# Autodesk Inventor assembly: Hose Assembly
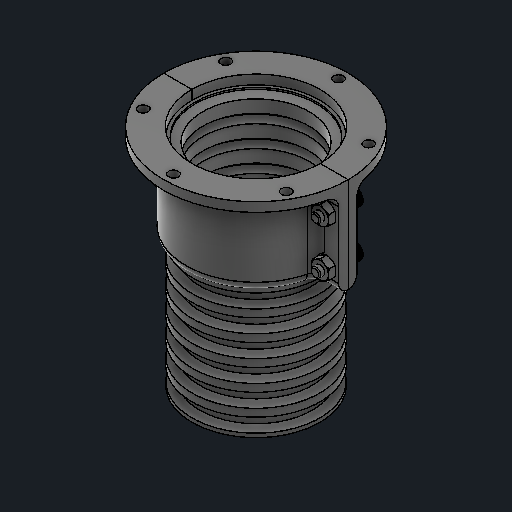
[picture p0: Inventor's stored thumbnail of the model, 512x512]
Saved by Autodesk Inventor 2026.2 (Build 302298000, 298)
## iProperties
Created: 2026-07-12
Part Number: Hose Assembly
Document SubType Name: Assembly
Designer: JoshuaEah
Author: JoshuaEah
## Documents named in this file (5)
- C:\Users\JoshuaEah\Documents\GitHub\Designed-Trinkets\Makera Carvera Air\Air Port\Hose Assembly.iam
- C:\Users\JoshuaEah\Documents\GitHub\Designed-Trinkets\Makera Carvera Air\Air Port\Vac Adapter.ipt
- C:\Users\JoshuaEah\Documents\GitHub\Designed-Trinkets\Makera Carvera Air\Air Port\40mm Vacuum Hose.ipt
- C:\Users\JoshuaEah\Documents\GitHub\Designed-Trinkets\Makera Carvera Air\Air Port\M3x10 SHCS.ipt
- C:\Users\JoshuaEah\Documents\GitHub\Designed-Trinkets\Makera Carvera Air\Air Port\M3x0.5 Hex Nut.ipt
## Components (11 placed, 4 different names)
1. Vac Adapter:1 — Insert:1, Insert:2, Insert:3, Insert:6, Insert:7, Insert:10, Insert:11
2. Vac Adapter:2 — Insert:1, Insert:2, Insert:4, Insert:5, Insert:8, Insert:9
3. 40mm Vacuum Hose:1 — Insert:3
4. M3x10 SHCS:1 — Insert:4
5. M3x10 SHCS:2 — Insert:5
6. M3x10 SHCS:3 — Insert:6
7. M3x10 SHCS:4 — Insert:7
8. M3x0.5 Hex Nut:1 — Insert:8
9. M3x0.5 Hex Nut:2 — Insert:9
10. M3x0.5 Hex Nut:3 — Insert:10
11. M3x0.5 Hex Nut:4 — Insert:11
## Relationships (11: Insert 11)
- Insert:1: Vac Adapter:1 ↔ Vac Adapter:2
- Insert:2: Vac Adapter:1 ↔ Vac Adapter:2
- Insert:3 (0.1 mm): Vac Adapter:1 ↔ 40mm Vacuum Hose:1
- Insert:4: Vac Adapter:2 ↔ M3x10 SHCS:1
- Insert:5: Vac Adapter:2 ↔ M3x10 SHCS:2
- Insert:6: Vac Adapter:1 ↔ M3x10 SHCS:3
- Insert:7: Vac Adapter:1 ↔ M3x10 SHCS:4
- Insert:8: Vac Adapter:2 ↔ M3x0.5 Hex Nut:1
- Insert:9: Vac Adapter:2 ↔ M3x0.5 Hex Nut:2
- Insert:10: Vac Adapter:1 ↔ M3x0.5 Hex Nut:3
- Insert:11: Vac Adapter:1 ↔ M3x0.5 Hex Nut:4
